# Autodesk Inventor assembly: arm asembaly
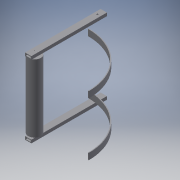
[picture p0: Inventor's stored thumbnail of the model, 180x180]
Saved by Autodesk Inventor 2016 (Build 200138000, 138)
## iProperties
Created: 2016-01-16
Part Number: arm asembaly
Document SubType Name: Assembly
Designer: Thariq
Author: Thariq
## Documents named in this file (5)
- C:\Users\Thariq\Documents\arm asembaly.iam
- C:\Users\Thariq\Documents\pickarm.ipt
- C:\Users\Thariq\Documents\rail.ipt
- C:\Users\Thariq\Documents\axel.ipt
- C:\Users\Thariq\Documents\roller.ipt
## Components (6 placed, 4 different names)
1. pickarm:1 — Mate:1, Mate:5, Flush:4, Mate:8
2. pickarm:2 — Mate:1, Mate:3, Mate:4, Flush:4, Mate:6, Flush:5
3. rail:1 — Mate:2, Flush:2, Flush:3, Mate:5
4. rail:2 — Mate:2, Flush:2, Flush:3, Mate:3, Mate:4
5. axel:1 — Mate:6, Flush:5, Mate:7
6. roller:1 — Mate:7, Mate:8
## Relationships (12: Mate 8, Flush 4)
- Mate:1 (279.4 mm): pickarm:1 ↔ pickarm:2
- Mate:2 (190.5 mm): rail:1 ↔ rail:2
- Flush:2: rail:1 ↔ rail:2
- Flush:3: rail:1 ↔ rail:2
- Mate:3 (19.05 mm): pickarm:2 ↔ rail:2
- Mate:4: pickarm:2 ↔ rail:2
- Mate:5: pickarm:1 ↔ rail:1
- Flush:4: pickarm:1 ↔ pickarm:2
- Mate:6: pickarm:2 ↔ axel:1
- Flush:5: pickarm:2 ↔ axel:1
- Mate:7: axel:1 ↔ roller:1
- Mate:8: pickarm:1 ↔ roller:1
